# Autodesk Inventor assembly: Freezer cabinet
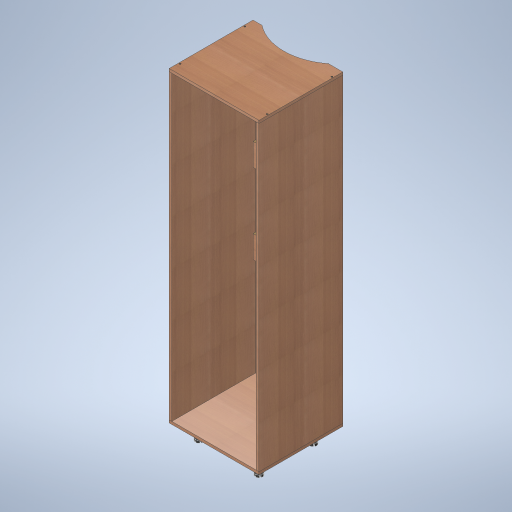
[picture p0: Inventor's stored thumbnail of the model, 512x512]
Saved by Autodesk Inventor 2024 (Build 280153000, 153)
## iProperties
RuleStatus: InUse
Created: 2017-01-31
Part Number: Freezer cabinet
Document SubType Name: Assembly
Designer: SvetlanaB
Author: SvetlanaB
## Documents named in this file (17)
- C:\W4INV 2024 Design\iBOX LIBRARY\Kitchen\Standing Cabinets\Freezer cabinet\Freezer cabinet.iam
- C:\W4INV 2024 Design\iBOX LIBRARY\Kitchen\Standing Cabinets\Freezer cabinet\Left panel.ipt
- C:\W4INV 2024 Design\iBOX LIBRARY\Kitchen\Standing Cabinets\Freezer cabinet\Top panel.ipt
- C:\W4INV 2024 Design\iBOX LIBRARY\Kitchen\Standing Cabinets\Freezer cabinet\Right panel.ipt
- C:\W4INV 2024 Design\iBOX LIBRARY\Kitchen\Standing Cabinets\Freezer cabinet\Bottom panel.ipt
- C:\W4INV 2024 Design\iBOX LIBRARY\Kitchen\Standing Cabinets\Freezer cabinet\Panel_1.ipt
- C:\W4INV 2024 Design\iBOX LIBRARY\Kitchen\Standing Cabinets\Freezer cabinet\Panel_2.ipt
- C:\W4INV 2024 Design\_LIBRARY\Supports and legs\Legs\ADJUSTABLE LEG\Adjustable leg  BT18 clip included.ipt
- C:\W4INV 2024 Design\_LIBRARY\Supports and legs\Legs\ADJUSTABLE LEG\Adjustable leg  BT18.ipt
- C:\W4INV 2024 Design\_LIBRARY\Fixed joints\Confirmat\CONFIRMAT\Confirmat L50 NB T18 PB T 18.ipt
- C:\W4INV 2024 Design\iBOX LIBRARY\Kitchen\Standing Cabinets\Freezer cabinet\Freezer cabinet.ipt
- C:\W4INV 2024 Design\_LIBRARY\Fixed joints\Minifix joint\MINIFIX D15 v2\Minifix D15 & Dowel L34 & Cap D15 PB T18 LH.ipt
- C:\W4INV 2024 Design\_LIBRARY\Fixed joints\Minifix joint\MINIFIX D15 v2\Minifix D15 & Dowel L34 & Cap D15 PB T18 RH.ipt
- C:\W4INV 2024 Design\_LIBRARY\Fixed joints\Confirmat\CONFIRMAT\Confirmat L50 & Cap D10 NB T18 PB T 18.ipt
- C:\W4INV 2023 Design\LIBRARY\Fixed joints\Confirmat\CONFIRMAT.ipt
- C:\W4INV 2023 Design\LIBRARY\Fixed joints\Minifix joint\MINIFIX D15 v2.ipt
- C:\W4INV 2023 Design\LIBRARY\Supports and legs\Legs\ADJUSTABLE LEG.ipt
## Components (23 placed, 13 different names)
1. @Skeleton
2. Left panel:1 — Flush:17, Pillar Board Side Plane:1, Pillar Board Side Plane:2, Pillar Board Side Plane:5, Pillar Board Side Plane:6, Nestled Board Plane:11, Nestled Board Plane:13
3. Top panel:1 — Nestled Board Plane:1, Nestled Board Plane:3, Nestled Board Plane:5, Nestled Board Plane:7
4. Right panel:1 — Flush:1, Flush:2, Flush:18, Pillar Board Side Plane:3, Pillar Board Side Plane:4, Pillar Board Side Plane:7, Pillar Board Side Plane:8, Nestled Board Plane:9, Nestled Board Plane:14
5. Bottom panel:1 — Flush:19, Flush:20, Bottom board Plane:1, Front (Angle) Plane:1, Bottom board Plane:2, Front (Angle) Plane:2, Bottom board Plane:3, Front (Angle) Plane:3, Bottom board Plane:4, Front (Angle) Plane:4, Nestled Board Plane:2, Nestled Board Plane:4, Nestled Board Plane:6, Nestled Board Plane:8
6. Panel_1:1 — Flush:3, Pillar Board Side Plane :1, Pillar Board Side Plane :2
7. Panel_2:1 — Flush:4, Pillar Board Side Plane :3, Pillar Board Side Plane :4
8. Adjustable leg  BT18 clip included:1 — Axis2 Plane:1, Axis Plane:13, Bottom board Plane:1, Front (Angle) Plane:1
9. Adjustable leg  BT18 clip included:2 — Axis2 Plane:2, Axis Plane:14, Bottom board Plane:2, Front (Angle) Plane:2
10. Adjustable leg  BT18:3 — Axis2 Plane:3, Axis Plane:15, Bottom board Plane:3, Front (Angle) Plane:3
11. Adjustable leg  BT18:4 — Axis2 Plane:4, Axis Plane:16, Bottom board Plane:4, Front (Angle) Plane:4
12. Confirmat L50 & Cap D10 NB T18 PB T 18:1 — Axis Plane:1, Pillar Board Side Plane:1, Nestled Board Plane:1
13. Confirmat L50 NB T18 PB T 18:2 — Axis Plane:2, Pillar Board Side Plane:2, Nestled Board Plane:2
14. Confirmat L50 NB T18 PB T 18:3 — Axis Plane:3, Pillar Board Side Plane:3, Nestled Board Plane:3
15. Confirmat L50 NB T18 PB T 18:4 — Axis Plane:4, Pillar Board Side Plane:4, Nestled Board Plane:4
16. Confirmat L50 NB T18 PB T 18:5 — Axis Plane:5, Pillar Board Side Plane:5, Nestled Board Plane:5
17. Confirmat L50 NB T18 PB T 18:6 — Axis Plane:6, Pillar Board Side Plane:6, Nestled Board Plane:6
18. Confirmat L50 NB T18 PB T 18:7 — Axis Plane:7, Pillar Board Side Plane:7, Nestled Board Plane:7
19. Confirmat L50 NB T18 PB T 18:8 — Axis Plane:8, Pillar Board Side Plane:8, Nestled Board Plane:8
20. Minifix D15 & Dowel L34 & Cap D15 PB T18 RH:1 — Nestled Board Plane:9, Pillar Board Side Plane :1, Axis Plane:9
21. Minifix D15 & Dowel L34 & Cap D15 PB T18 LH:2 — Nestled Board Plane:11, Pillar Board Side Plane :2, Axis Plane:11
22. Minifix D15 & Dowel L34 & Cap D15 PB T18 RH:3 — Nestled Board Plane:13, Pillar Board Side Plane :3, Axis Plane:17
23. Minifix D15 & Dowel L34 & Cap D15 PB T18 LH:4 — Nestled Board Plane:14, Pillar Board Side Plane :4, Axis Plane:18
## Relationships (60: Mate 36, Flush 20, Angle 4)
- Flush:1 (-64 mm): Right panel:1
- Flush:2 (-64 mm): Right panel:1
- Flush:3 (-50 mm): Panel_1:1
- Flush:4 (-50 mm): Panel_2:1
- Flush:17 (-100 mm): Left panel:1
- Flush:18 (-100 mm): Right panel:1
- Flush:19 (-100 mm): Bottom panel:1
- Flush:20 (-100 mm): Bottom panel:1
- Axis2 Plane:1 [Mate]: Adjustable leg  BT18 clip included:1
- Axis Plane:13 [Mate]: Adjustable leg  BT18 clip included:1
- Bottom board Plane:1 [Mate]: Bottom panel:1 ↔ Adjustable leg  BT18 clip included:1
- Front (Angle) Plane:1 [Angle] (0 deg): Bottom panel:1 ↔ Adjustable leg  BT18 clip included:1
- Axis2 Plane:2 [Mate]: Adjustable leg  BT18 clip included:2
- Axis Plane:14 [Mate]: Adjustable leg  BT18 clip included:2
- Bottom board Plane:2 [Mate]: Bottom panel:1 ↔ Adjustable leg  BT18 clip included:2
- Front (Angle) Plane:2 [Angle] (0 deg): Bottom panel:1 ↔ Adjustable leg  BT18 clip included:2
- Axis2 Plane:3 [Mate]: Adjustable leg  BT18:3
- Axis Plane:15 [Mate]: Adjustable leg  BT18:3
- Bottom board Plane:3 [Mate]: Bottom panel:1 ↔ Adjustable leg  BT18:3
- Front (Angle) Plane:3 [Angle] (0 deg): Bottom panel:1 ↔ Adjustable leg  BT18:3
- Axis2 Plane:4 [Mate]: Adjustable leg  BT18:4
- Axis Plane:16 [Mate]: Adjustable leg  BT18:4
- Bottom board Plane:4 [Mate]: Bottom panel:1 ↔ Adjustable leg  BT18:4
- Front (Angle) Plane:4 [Angle] (0 deg): Bottom panel:1 ↔ Adjustable leg  BT18:4
- Axis Plane:1 [Mate]: Confirmat L50 & Cap D10 NB T18 PB T 18:1
- Pillar Board Side Plane:1 [Mate] (-9 mm): Left panel:1 ↔ Confirmat L50 & Cap D10 NB T18 PB T 18:1
- Nestled Board Plane:1 [Flush]: Top panel:1 ↔ Confirmat L50 & Cap D10 NB T18 PB T 18:1
- Axis Plane:2 [Mate]: Confirmat L50 NB T18 PB T 18:2
- Pillar Board Side Plane:2 [Mate] (-9 mm): Left panel:1 ↔ Confirmat L50 NB T18 PB T 18:2
- Nestled Board Plane:2 [Flush]: Bottom panel:1 ↔ Confirmat L50 NB T18 PB T 18:2
- Axis Plane:3 [Mate]: Confirmat L50 NB T18 PB T 18:3
- Pillar Board Side Plane:3 [Mate] (-9 mm): Right panel:1 ↔ Confirmat L50 NB T18 PB T 18:3
- Nestled Board Plane:3 [Flush]: Top panel:1 ↔ Confirmat L50 NB T18 PB T 18:3
- Axis Plane:4 [Mate]: Confirmat L50 NB T18 PB T 18:4
- Pillar Board Side Plane:4 [Mate] (-9 mm): Right panel:1 ↔ Confirmat L50 NB T18 PB T 18:4
- Nestled Board Plane:4 [Flush]: Bottom panel:1 ↔ Confirmat L50 NB T18 PB T 18:4
- Axis Plane:5 [Mate]: Confirmat L50 NB T18 PB T 18:5
- Pillar Board Side Plane:5 [Mate] (-9 mm): Left panel:1 ↔ Confirmat L50 NB T18 PB T 18:5
- Nestled Board Plane:5 [Flush]: Top panel:1 ↔ Confirmat L50 NB T18 PB T 18:5
- Axis Plane:6 [Mate]: Confirmat L50 NB T18 PB T 18:6
- Pillar Board Side Plane:6 [Mate] (-9 mm): Left panel:1 ↔ Confirmat L50 NB T18 PB T 18:6
- Nestled Board Plane:6 [Flush]: Bottom panel:1 ↔ Confirmat L50 NB T18 PB T 18:6
- Axis Plane:7 [Mate]: Confirmat L50 NB T18 PB T 18:7
- Pillar Board Side Plane:7 [Mate] (-9 mm): Right panel:1 ↔ Confirmat L50 NB T18 PB T 18:7
- Nestled Board Plane:7 [Flush]: Top panel:1 ↔ Confirmat L50 NB T18 PB T 18:7
- Axis Plane:8 [Mate]: Confirmat L50 NB T18 PB T 18:8
- Pillar Board Side Plane:8 [Mate] (-9 mm): Right panel:1 ↔ Confirmat L50 NB T18 PB T 18:8
- Nestled Board Plane:8 [Flush]: Bottom panel:1 ↔ Confirmat L50 NB T18 PB T 18:8
- Nestled Board Plane:9 [Mate]: Right panel:1 ↔ Minifix D15 & Dowel L34 & Cap D15 PB T18 RH:1
- Pillar Board Side Plane :1 [Flush] (18 mm): Panel_1:1 ↔ Minifix D15 & Dowel L34 & Cap D15 PB T18 RH:1
- Axis Plane:9 [Mate]: Minifix D15 & Dowel L34 & Cap D15 PB T18 RH:1
- Nestled Board Plane:11 [Mate]: Left panel:1 ↔ Minifix D15 & Dowel L34 & Cap D15 PB T18 LH:2
- Pillar Board Side Plane :2 [Flush] (18 mm): Panel_1:1 ↔ Minifix D15 & Dowel L34 & Cap D15 PB T18 LH:2
- Axis Plane:11 [Mate]: Minifix D15 & Dowel L34 & Cap D15 PB T18 LH:2
- Nestled Board Plane:13 [Mate]: Left panel:1 ↔ Minifix D15 & Dowel L34 & Cap D15 PB T18 RH:3
- Pillar Board Side Plane :3 [Flush] (18 mm): Panel_2:1 ↔ Minifix D15 & Dowel L34 & Cap D15 PB T18 RH:3
- Axis Plane:17 [Mate]: Minifix D15 & Dowel L34 & Cap D15 PB T18 RH:3
- Nestled Board Plane:14 [Mate]: Right panel:1 ↔ Minifix D15 & Dowel L34 & Cap D15 PB T18 LH:4
- Pillar Board Side Plane :4 [Flush] (18 mm): Panel_2:1 ↔ Minifix D15 & Dowel L34 & Cap D15 PB T18 LH:4
- Axis Plane:18 [Mate]: Minifix D15 & Dowel L34 & Cap D15 PB T18 LH:4
## Named parameters: Panel_thickness = 18 mm
